# Autodesk Inventor assembly: CanSat
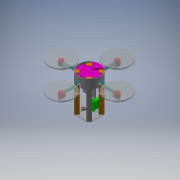
[picture p0: Inventor's stored thumbnail of the model, 180x180]
Saved by Autodesk Inventor 2018 (Build 220112000, 112)
## iProperties
Created: 2017-12-31
Part Number: CanSat
Document SubType Name: Assembly
Designer: suchanek
Author: suchanek
## Documents named in this file (16)
- C:\Users\sucha\programming\CanSat\Schematics\Model\CanSat.iam
- C:\Users\sucha\programming\CanSat\Schematics\Model\Hull.ipt
- C:\Users\sucha\programming\CanSat\Schematics\Model\Arm.ipt
- C:\Users\sucha\programming\CanSat\Schematics\Model\Motor.ipt
- C:\Users\sucha\programming\CanSat\Schematics\Model\Rotor.ipt
- C:\Users\sucha\programming\CanSat\Schematics\Model\Battery_small.ipt
- C:\Users\sucha\programming\CanSat\Schematics\Model\Servo.ipt
- C:\Users\sucha\programming\CanSat\Schematics\Model\Spring.ipt
- C:\Users\sucha\programming\CanSat\Schematics\Model\Servo_bit.ipt
- C:\Users\sucha\programming\CanSat\Schematics\Model\Scraper.ipt
- C:\Users\sucha\programming\CanSat\Schematics\Model\Petri.ipt
- C:\Users\sucha\programming\CanSat\Schematics\Model\Axel.ipt
- C:\Users\sucha\programming\CanSat\Schematics\Model\Circuit.ipt
- C:\Users\sucha\programming\CanSat\Schematics\Model\Flight_controler.ipt
- C:\Users\sucha\programming\CanSat\Schematics\Model\HGLRC Micro 13A 4in1 BLHeli_S.ipt
- C:\Users\sucha\programming\CanSat\Schematics\Model\SIM808 Module GSM GPRS GPS Breakout Board SIM808 for Arduino Raspberry.ipt
## Components (43 placed, 15 different names)
1. Hull:1 — Cylindrical:1, Mate:2, Mate:3, Mate:13, Mate:14, Mate:15, Cylindrical:2, Mate:16, Mate:17, Mate:18, Mate:19, Mate:20, Flush:1, Slider:1, Planar:1, Cylindrical:3, Mate:22, Cylindrical:5, Mate:23, Cylindrical:7, Mate:24, Cylindrical:9, Mate:25, Mate:26, Mate:27, Mate:28, Angle:1, Angle:2, Mate:29, Angle:3, Angle:4, Rotational:25, Mate:30, Rigid:9, Rotational:26
2. Arm:1 — Rigid:5, Mate:24, Cylindrical:10, Angle:1
3. Arm:2 — Rigid:4, Mate:23, Cylindrical:8, Angle:3
4. Arm:3 — Rigid:3, Mate:22, Cylindrical:6, Angle:4
5. Arm:4 — Rigid:2, Cylindrical:4, Angle:2, Mate:29
6. Motor:1 — Rigid:2, Rotational:8
7. Motor:2 — Rigid:3, Rotational:9
8. Motor:3 — Rigid:4, Rotational:11
9. Motor:4 — Rigid:5, Rotational:10
10. Rotor:1 — Rotational:8
11. Rotor:2 — Rotational:10
12. Rotor:3 — Rotational:9
13. Rotor:4 — Rotational:11
14. Battery_small:1 — Cylindrical:1, Rotational:12, Mate:1, Mate:2, Rotational:13
15. Battery_small:2 — Rotational:12, Mate:1
16. Battery_small:3 — Rotational:13, Mate:3, Rotational:14, Mate:4
17. Battery_small:4 — Rotational:18, Mate:9, Rotational:22, Cylindrical:2
18. Battery_small:5 — Rotational:18, Mate:9
19. Battery_small:6 — Rotational:17, Mate:7, Mate:11
20. Battery_small:7 — Rotational:14, Mate:4
21. Battery_small:8 — Rotational:16, Mate:6, Mate:12
22. Battery_small:9 — Rotational:19, Mate:8
23. Battery_small:10 — Rotational:19, Mate:8, Rotational:23, Mate:19, Mate:20
24. Battery_small:11 — Rotational:20, Mate:10, Rotational:23, Mate:18
25. Battery_small:12 — Rotational:20, Mate:10
26. Battery_small:13 — Mate:5, Rotational:15
27. Battery_small:14 — Rotational:17, Mate:7, Mate:11, Rotational:22, Mate:16, Mate:17
28. Battery_small:15 — Mate:5, Rotational:15, Rotational:21, Mate:15
29. Battery_small:16 — Rotational:16, Mate:6, Mate:12, Rotational:21, Mate:13, Mate:14
30. Servo:1 — Flush:1, Slider:1, Rotational:24
31. Spring:1 — Rigid:6, Rigid:7
32. Servo_bit:1 — Rotational:24, Rigid:6
33. Scraper:1 — Rigid:7
34. Petri:1 — Planar:1
35. Axel:1 — Cylindrical:7, Cylindrical:8, Mate:28
36. Axel:2 — Cylindrical:5, Cylindrical:6, Mate:25
37. Axel:3 — Cylindrical:9, Cylindrical:10, Mate:27
38. Axel:4 — Cylindrical:3, Cylindrical:4, Mate:26
39. Circuit:1 — Rotational:25, Mate:30, Rigid:8
40. Flight_controler:1 — Rigid:8
41. HGLRC Micro 13A 4in1 BLHeli_S:1
42. HGLRC Micro 13A 4in1 BLHeli_S:2 — Rigid:9
43. SIM808 Module GSM GPRS GPS Breakout Board SIM808 for Arduino Raspberry:1 — Rotational:26
## Relationships (73: Mate 29, RevoluteJoint 19, CylindricalJoint 10, WeldJoint 8, Angle 4, Flush 1, TranslationJoint 1, PlanarJoint 1)
- Rigid:2 [WeldJoint]: Arm:4 ↔ Motor:1
- Rotational:8 [RevoluteJoint]: Motor:1 ↔ Rotor:1
- Rigid:3 [WeldJoint]: Arm:3 ↔ Motor:2
- Rotational:9 [RevoluteJoint]: Motor:2 ↔ Rotor:3
- Rigid:4 [WeldJoint]: Arm:2 ↔ Motor:3
- Rigid:5 [WeldJoint]: Arm:1 ↔ Motor:4
- Rotational:10 [RevoluteJoint]: Motor:4 ↔ Rotor:2
- Rotational:11 [RevoluteJoint]: Motor:3 ↔ Rotor:4
- Cylindrical:1: Hull:1 ↔ Battery_small:1
- Rotational:12 [RevoluteJoint] (5 mm): Battery_small:1 ↔ Battery_small:2
- Mate:1: Battery_small:1 ↔ Battery_small:2
- Mate:2: Hull:1 ↔ Battery_small:1
- Rotational:13 [RevoluteJoint]: Battery_small:1 ↔ Battery_small:3
- Mate:3: Hull:1 ↔ Battery_small:3
- Rotational:14 [RevoluteJoint] (5 mm): Battery_small:3 ↔ Battery_small:7
- Mate:4: Battery_small:3 ↔ Battery_small:7
- Mate:5: Battery_small:13 ↔ Battery_small:15
- Rotational:15 [RevoluteJoint] (5 mm): Battery_small:13 ↔ Battery_small:15
- Rotational:16 [RevoluteJoint] (5 mm): Battery_small:8 ↔ Battery_small:16
- Rotational:17 [RevoluteJoint] (5 mm): Battery_small:6 ↔ Battery_small:14
- Rotational:18 [RevoluteJoint] (5 mm): Battery_small:4 ↔ Battery_small:5
- Rotational:19 [RevoluteJoint] (5 mm): Battery_small:9 ↔ Battery_small:10
- Mate:6: Battery_small:8 ↔ Battery_small:16
- Mate:7: Battery_small:6 ↔ Battery_small:14
- Rotational:20 [RevoluteJoint] (5 mm): Battery_small:11 ↔ Battery_small:12
- Mate:8: Battery_small:9 ↔ Battery_small:10
- Mate:9: Battery_small:4 ↔ Battery_small:5
- Mate:10: Battery_small:11 ↔ Battery_small:12
- Mate:11: Battery_small:6 ↔ Battery_small:14
- Mate:12: Battery_small:8 ↔ Battery_small:16
- Rotational:21 [RevoluteJoint]: Battery_small:15 ↔ Battery_small:16
- Rotational:22 [RevoluteJoint]: Battery_small:4 ↔ Battery_small:14
- Rotational:23 [RevoluteJoint]: Battery_small:10 ↔ Battery_small:11
- Mate:13: Hull:1 ↔ Battery_small:16
- Mate:14: Hull:1 ↔ Battery_small:16
- Mate:15: Hull:1 ↔ Battery_small:15
- Cylindrical:2: Hull:1 ↔ Battery_small:4
- Mate:16: Hull:1 ↔ Battery_small:14
- Mate:17: Hull:1 ↔ Battery_small:14
- Mate:18: Hull:1 ↔ Battery_small:11
- Mate:19: Hull:1 ↔ Battery_small:10
- Mate:20: Hull:1 ↔ Battery_small:10
- Flush:1: Hull:1 ↔ Servo:1
- Slider:1 [TranslationJoint]: Hull:1 ↔ Servo:1
- Rotational:24 [RevoluteJoint]: Servo:1 ↔ Servo_bit:1
- Rigid:6 [WeldJoint]: Spring:1 ↔ Servo_bit:1
- Rigid:7 [WeldJoint]: Spring:1 ↔ Scraper:1
- Planar:1: Hull:1 ↔ Petri:1
- Cylindrical:3: Hull:1 ↔ Axel:4
- Cylindrical:4: Arm:4 ↔ Axel:4
- Mate:22: Hull:1 ↔ Arm:3
- Cylindrical:5: Hull:1 ↔ Axel:2
- Cylindrical:6: Arm:3 ↔ Axel:2
- Mate:23: Hull:1 ↔ Arm:2
- Cylindrical:7: Hull:1 ↔ Axel:1
- Cylindrical:8: Arm:2 ↔ Axel:1
- Mate:24: Hull:1 ↔ Arm:1
- Cylindrical:9: Hull:1 ↔ Axel:3
- Cylindrical:10: Arm:1 ↔ Axel:3
- Mate:25: Hull:1 ↔ Axel:2
- Mate:26: Hull:1 ↔ Axel:4
- Mate:27: Hull:1 ↔ Axel:3
- Mate:28: Hull:1 ↔ Axel:1
- Angle:1 (0 deg): Hull:1 ↔ Arm:1
- Angle:2 (0 deg): Hull:1 ↔ Arm:4
- Mate:29: Hull:1 ↔ Arm:4
- Angle:3 (0 deg): Hull:1 ↔ Arm:2
- Angle:4 (0 deg): Hull:1 ↔ Arm:3
- Rotational:25 [RevoluteJoint] (5 mm): Hull:1 ↔ Circuit:1
- Mate:30 (0.5 mm): Hull:1 ↔ Circuit:1
- Rigid:8 [WeldJoint]: Circuit:1 ↔ Flight_controler:1
- Rigid:9 [WeldJoint]: Hull:1 ↔ HGLRC Micro 13A 4in1 BLHeli_S:2
- Rotational:26 [RevoluteJoint]: Hull:1 ↔ SIM808 Module GSM GPRS GPS Breakout Board SIM808 for Arduino Raspberry:1
